# Autodesk Inventor assembly: mr-20cnb_mrs20-1200_0
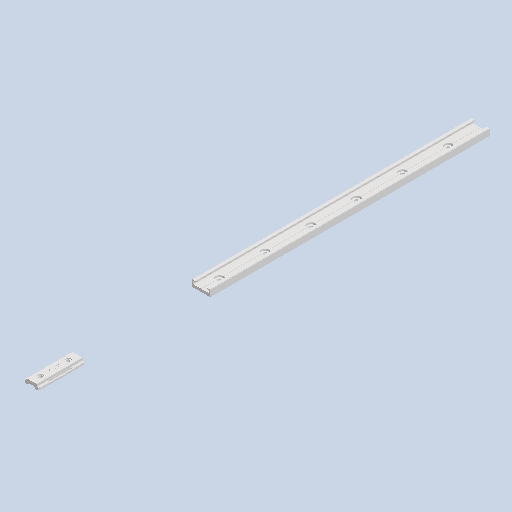
[picture p0: Inventor's stored thumbnail of the model, 512x512]
Saved by Autodesk Inventor 2024.1 (Build 281209000, 209)
## iProperties
Created: 2020-09-01
Part Number: mr-20cnb_mrs20-1200_0
Description: STEP AP203
Document SubType Name: Assembly
Designer: morita masato
Sending System: SolidWorks 2017
Preprocessor: SwSTEP 2.0
Title: MR-20CNB_MRS20-1200_0.step
Revision Number: ANY
## Documents named in this file (3)
- C:\Users\haruy\OneDrive - Kyushu University\KURT_工房共有\2023~2024\ハード\CAD\2024NHK\000_parts\スライダー\mr-20cnb_mrs20-1200_0.iam
- C:\Users\haruy\OneDrive - Kyushu University\KURT_工房共有\2023~2024\ハード\CAD\2024NHK\000_parts\スライダー\MR-20CNB.iam
- C:\Users\haruy\OneDrive - Kyushu University\KURT_工房共有\2023~2024\ハード\CAD\2024NHK\000_parts\スライダー\mrs20-1200.ipt
## Components (2 placed, 2 different names)
1. MR-20CNB_1 [sub-assembly] — メイト:1, メイト:2, メイト:3
2. mrs20-1200_2 — メイト:1, メイト:2, メイト:3
## Relationships (3: Mate 3)
- メイト:1 [Mate]: MR-20CNB_1 ↔ mrs20-1200_2
- メイト:2 [Mate] (0.1 mm): MR-20CNB_1 ↔ mrs20-1200_2
- メイト:3 [Mate] (0.1 mm): MR-20CNB_1 ↔ mrs20-1200_2
